# Autodesk Inventor assembly: face
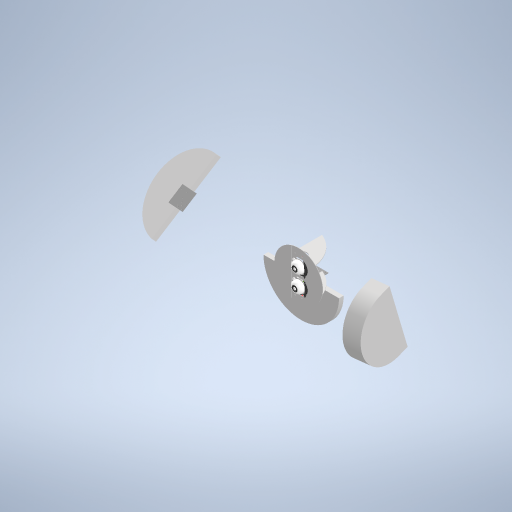
[picture p0: Inventor's stored thumbnail of the model, 512x512]
Saved by Autodesk Inventor 2023.2 (Build 272271030, 271C)
## iProperties
Created: 2024-01-26
Part Number: face
Document SubType Name: Assembly
Designer: I9232
Author: I9232
## Documents named in this file (9)
- D:\!project\fox_n_crow_construction\crow\face\face.iam
- D:\!project\fox_n_crow_construction\crow\face\Сборка глаза вороны.iam
- C:\Users\I9232\OneDrive\Рабочий стол\Проект\Модели\Ворона\Деталь1.ipt
- D:\!project\fox_n_crow_construction\crow\face\Платформа для крыльев лево.ipt
- D:\!project\fox_n_crow_construction\crow\face\Платформа для крыльев право.ipt
- C:\Users\I9232\OneDrive\Рабочий стол\Проект\Модели\Ворона\Крылья\step\Сыр\Сыр.ipt
- C:\Users\I9232\OneDrive\Рабочий стол\Проект\Модели\Ворона\Крылья\step\Веер\Веер.ipt
- D:\!project\fox_n_crow_construction\crow\face\боковые стороны головы.ipt
- D:\!project\fox_n_crow_construction\crow\face\боковые стороны головы_MIR.ipt
## Components (9 placed, 8 different names)
1. Сборка глаза вороны:1 [sub-assembly] — Заподлицо:1
2. Платформа глаз — Заподлицо:1, Заподлицо:5, Совмещение:5, Совмещение:6, Совмещение:7
3. Платформа для крыльев лево:1 — Совмещение:3, Совмещение:4
4. Платформа для крыльев право:1 — Заподлицо:2, Совмещение:1, Совмещение:2, Заподлицо:3
5. Сыр:1
6. Веер:1 — Заподлицо:2, Совмещение:1, Совмещение:2, Заподлицо:3
7. Веер:2 — Совмещение:3, Совмещение:4
8. боковые стороны головы:1 — Заподлицо:5, Совмещение:7
9. боковые стороны головы_MIR:1 — Совмещение:5, Совмещение:6
## Relationships (11: Mate 7, Flush 4)
- Заподлицо:1 [Flush]: Сборка глаза вороны:1 ↔ Платформа глаз
- Заподлицо:2 [Flush]: Платформа для крыльев право:1 ↔ Веер:1
- Совмещение:1 [Mate]: Платформа для крыльев право:1 ↔ Веер:1
- Совмещение:2 [Mate]: Платформа для крыльев право:1 ↔ Веер:1
- Заподлицо:3 [Flush]: Платформа для крыльев право:1 ↔ Веер:1
- Совмещение:3 [Mate]: Платформа для крыльев лево:1 ↔ Веер:2
- Совмещение:4 [Mate]: Платформа для крыльев лево:1 ↔ Веер:2
- Заподлицо:5 [Flush]: Платформа глаз ↔ боковые стороны головы:1
- Совмещение:5 [Mate]: Платформа глаз ↔ боковые стороны головы_MIR:1
- Совмещение:6 [Mate]: Платформа глаз ↔ боковые стороны головы_MIR:1
- Совмещение:7 [Mate]: Платформа глаз ↔ боковые стороны головы:1
